# Autodesk Inventor assembly: Engrenagens 2
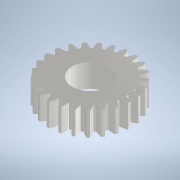
[picture p0: Inventor's stored thumbnail of the model, 180x180]
Saved by Autodesk Inventor 2021 (Build 250183000, 183)
## iProperties
Created: 2021-07-23
Part Number: Engrenagens 2
Document SubType Name: Assembly
Designer: Giovanni
Author: Giovanni
## Documents named in this file (2)
- C:\Users\irineu\Documents\Inventor\MotorRadial7\Engrenagens 2.iam
- C:\Users\irineu\Documents\Inventor\MotorRadial7\Engrenagens 2\Design Accelerator\Engrenagens retas1.iam
## Components (1 placed, 1 different names)
1. Engrenagens retas:1 [sub-assembly] — Coincidente:1, Coincidente:2, Alinhado:1
## Relationships (3: Mate 2, Flush 1)
- Coincidente:1 [Mate]: Engrenagens retas:1
- Coincidente:2 [Mate]: Engrenagens retas:1
- Alinhado:1 [Flush]: Engrenagens retas:1
